# Autodesk Inventor assembly: ABD_Version_0.1_leftleg
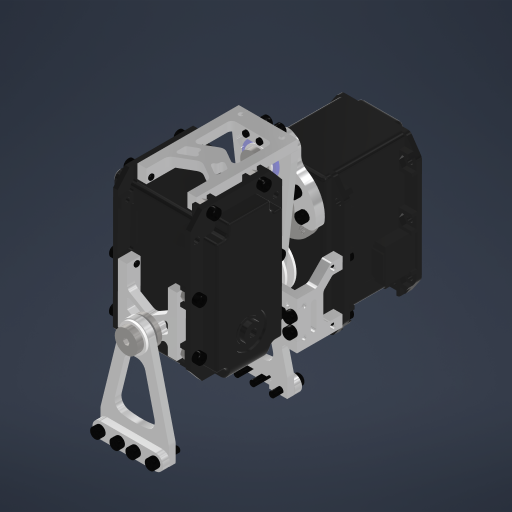
[picture p0: Inventor's stored thumbnail of the model, 512x512]
Saved by Autodesk Inventor 2024 (Build 280153000, 153)
## iProperties
Created: 2024-01-23
Part Number: ABD_Version_0.1_leftleg
Document SubType Name: Assembly
Designer: ASUS
Mass: 357.136 g
Surface Area: 604.848 cm^2
Volume: 181.423 cm^3
Density: 1.96853 g/cm^3
Author: ASUS
## Documents named in this file (11)
- C:\Users\ASUS\Desktop\Anti_Backlash_Structure_OP\v3_Frame\ABD_V3_Left_OP.iam
- C:\Users\ASUS\Desktop\Anti_Backlash_Structure_OP\v3_Frame\Roll_Fixation_Set.iam
- C:\Users\ASUS\Desktop\Anti_Backlash_Structure_OP\v3_Frame\ABD_MX_64_Roll_Fixation_Set.iam
- C:\Users\ASUS\Desktop\Anti_Backlash_Structure_OP\v3_Frame\ABD_MX_64_Slider_Fixation_Set_Right2Horn.iam
- C:\Users\ASUS\Desktop\Anti_Backlash_Structure_OP\v3_Frame\ABD_Slider_Set_v3.iam
- C:\Users\ASUS\Desktop\Anti_Backlash_Structure_OP\MISUMI\C-WSSA12-4-2.ipt
- C:\Users\ASUS\Desktop\Anti_Backlash_Structure_OP\MISUMI\TT-0612-10.ipt
- C:\Users\ASUS\Desktop\Anti_Backlash_Structure_OP\MISUMI\LED-0606.ipt
- C:\Users\ASUS\Desktop\Anti_Backlash_Structure_OP\v3_Frame\Ubber_Washer_1.5mm.ipt
- C:\Users\ASUS\Desktop\Anti_Backlash_Structure_OP\MISUMI\DBB4-8-5.ipt
- C:\Users\ASUS\Desktop\Anti_Backlash_Structure_OP\MISUMI\TT-0612-5.ipt
## Components (10 placed, 10 different names)
1. Roll_Fixation_Set:1 [sub-assembly] — 삽입:4, 삽입:5, 메이트:6, 각도:1
2. ABD_MX_64_Roll_Fixation_Set:1 [sub-assembly] — 메이트:2, 메이트:3, 삽입:5, 각도:1
3. ABD_MX_64_Slider_Fixation_Set_Right2Horn:1 [sub-assembly] — 삽입:4, 메이트:2, 메이트:3, 메이트:4, 메이트:5
4. C-WSSA12-4-2:1 — 삽입:7, 삽입:8
5. TT-0612-10:1 — 삽입:7, 삽입:10
6. ABD_Slider_Set_v3:1 [sub-assembly] — 메이트:6, 삽입:10
7. LED-0606:1 — 삽입:8, 삽입:9, 메이트:5
8. Ubber_Washer_1.5mm:1 — 삽입:9, 메이트:4, 삽입:11
9. TT-0612-5:1 — 삽입:11, 삽입:12
10. DBB4-8-5:1 — 삽입:12
## Relationships (14: Insert 8, Mate 5, Angle 1)
- 삽입:4 [Insert]: Roll_Fixation_Set:1 ↔ ABD_MX_64_Slider_Fixation_Set_Right2Horn:1
- 메이트:2 [Mate] (0.05 mm): ABD_MX_64_Roll_Fixation_Set:1 ↔ ABD_MX_64_Slider_Fixation_Set_Right2Horn:1
- 메이트:3 [Mate]: ABD_MX_64_Roll_Fixation_Set:1 ↔ ABD_MX_64_Slider_Fixation_Set_Right2Horn:1
- 삽입:5 [Insert]: Roll_Fixation_Set:1 ↔ ABD_MX_64_Roll_Fixation_Set:1
- 삽입:7 [Insert]: C-WSSA12-4-2:1 ↔ TT-0612-10:1
- 삽입:8 [Insert]: C-WSSA12-4-2:1 ↔ LED-0606:1
- 삽입:9 [Insert]: LED-0606:1 ↔ Ubber_Washer_1.5mm:1
- 메이트:4 [Mate]: ABD_MX_64_Slider_Fixation_Set_Right2Horn:1 ↔ Ubber_Washer_1.5mm:1
- 메이트:5 [Mate] (0.025 mm): ABD_MX_64_Slider_Fixation_Set_Right2Horn:1 ↔ LED-0606:1
- 메이트:6 [Mate]: Roll_Fixation_Set:1 ↔ ABD_Slider_Set_v3:1
- 삽입:10 [Insert]: TT-0612-10:1 ↔ ABD_Slider_Set_v3:1
- 각도:1 [Angle] (0 deg): Roll_Fixation_Set:1 ↔ ABD_MX_64_Roll_Fixation_Set:1
- 삽입:11 [Insert]: Ubber_Washer_1.5mm:1 ↔ TT-0612-5:1
- 삽입:12 [Insert]: TT-0612-5:1 ↔ DBB4-8-5:1
